# Autodesk Inventor assembly: LifterRight
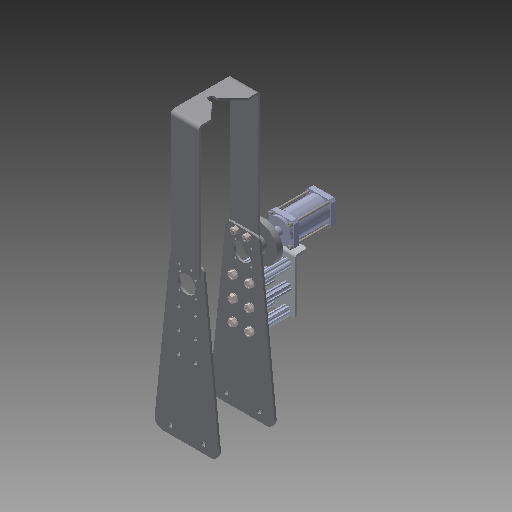
[picture p0: Inventor's stored thumbnail of the model, 512x512]
Saved by Autodesk Inventor 2017 (Build 210142000, 142)
## iProperties
Created: 2017-02-09
Part Number: LifterRight
Document SubType Name: Assembly
Designer: kingb
Author: kingb
## Documents named in this file (10)
- C:\Users\kingb\Desktop\CAD\LifterRight.iam
- C:\Users\kingb\Desktop\CAD\lifterMountMetal.ipt
- C:\Users\kingb\Desktop\CAD\am-2954 AM14U2 2x3 Hole Bracket.ipt
- C:\Users\kingb\Desktop\CAD\am-2878+Banebots+P60+256-11(Fixed).iam
- C:\Users\kingb\Desktop\CAD\newCoupler.ipt
- C:\Users\kingb\Desktop\CAD\Churro 3375.ipt
- C:\Users\kingb\Desktop\CAD\guidebar.ipt
- C:\Users\kingb\Desktop\CAD\10-32x0500_shcs_HX-SHCS 0.19-32x1.375x1-C.ipt
- C:\Users\kingb\Desktop\CAD\FHTS 0.25-20-0.75_FHTS 0.25-20-G-0.75-C.ipt
- C:\Users\kingb\Desktop\CAD\10-32 Nylock Nut.ipt
## Components (30 placed, 9 different names)
1. lifterMountMetal:1 — Mate:5, Mate:6, Insert:12, Insert:14, Insert:15, Insert:16, Insert:17, Insert:26, Insert:27, Mate:11, Mate:12, Mate:13
2. am-2954 AM14U2 2x3 Hole Bracket:1 — Mate:2, Flush:1, Mate:3, Insert:4, Insert:5, Insert:6, Insert:7, Insert:8, Insert:9, Insert:10, Insert:11, Insert:18, Insert:19, Insert:20, Insert:21, Insert:22, Insert:23
3. am-2878+Banebots+P60+256-11(Fixed):1 [sub-assembly] — Mate:2, Flush:1, Mate:3, Angle:2, Mate:13, Mate:14, Mate:15
4. newCoupler:1 — Mate:14, Mate:15
5. Churro 3375:1 — Insert:7
6. Churro 3375:2 — Insert:5
7. Churro 3375:3 — Insert:4, Mate:5
8. Churro 3375:5 — Insert:6
9. guidebar:1 — Mate:6, Angle:2, Insert:24, Insert:25, Insert:28, Insert:29, Mate:11, Mate:12
10. Churro 3375:6 — Insert:9
11. Churro 3375:7 — Insert:8
12. 10-32x0500_shcs_HX-SHCS 0.19-32x1.375x1-C:1 — Insert:10
13. 10-32x0500_shcs_HX-SHCS 0.19-32x1.375x1-C:2 — Insert:11
14. FHTS 0.25-20-0.75_FHTS 0.25-20-G-0.75-C:1 — Insert:20
15. FHTS 0.25-20-0.75_FHTS 0.25-20-G-0.75-C:2 — Insert:21
16. FHTS 0.25-20-0.75_FHTS 0.25-20-G-0.75-C:3 — Insert:23
17. FHTS 0.25-20-0.75_FHTS 0.25-20-G-0.75-C:4 — Insert:22
18. FHTS 0.25-20-0.75_FHTS 0.25-20-G-0.75-C:5 — Insert:18
19. FHTS 0.25-20-0.75_FHTS 0.25-20-G-0.75-C:6 — Insert:19
20. FHTS 0.25-20-0.75_FHTS 0.25-20-G-0.75-C:7 — Insert:16
21. FHTS 0.25-20-0.75_FHTS 0.25-20-G-0.75-C:8 — Insert:17
22. FHTS 0.25-20-0.75_FHTS 0.25-20-G-0.75-C:9 — Insert:14
23. FHTS 0.25-20-0.75_FHTS 0.25-20-G-0.75-C:10 — Insert:15
24. FHTS 0.25-20-0.75_FHTS 0.25-20-G-0.75-C:11
25. FHTS 0.25-20-0.75_FHTS 0.25-20-G-0.75-C:12 — Insert:12
26. 10-32x0500_shcs_HX-SHCS 0.19-32x1.375x1-C:3 — Insert:24
27. 10-32x0500_shcs_HX-SHCS 0.19-32x1.375x1-C:4 — Insert:25
28. 10-32 Nylock Nut:1 — Insert:27
29. 10-32 Nylock Nut:2 — Insert:26
30. lifterMountMetal:2 — Insert:28, Insert:29
## Relationships (36: Insert 25, Mate 9, Flush 1, Angle 1)
- Mate:2: am-2954 AM14U2 2x3 Hole Bracket:1 ↔ am-2878+Banebots+P60+256-11(Fixed):1
- Flush:1 (-6.35 mm): am-2954 AM14U2 2x3 Hole Bracket:1 ↔ am-2878+Banebots+P60+256-11(Fixed):1
- Mate:3: am-2954 AM14U2 2x3 Hole Bracket:1 ↔ am-2878+Banebots+P60+256-11(Fixed):1
- Insert:4: am-2954 AM14U2 2x3 Hole Bracket:1 ↔ Churro 3375:3
- Insert:5: am-2954 AM14U2 2x3 Hole Bracket:1 ↔ Churro 3375:2
- Mate:5: lifterMountMetal:1 ↔ Churro 3375:3
- Insert:6: am-2954 AM14U2 2x3 Hole Bracket:1 ↔ Churro 3375:5
- Insert:7: am-2954 AM14U2 2x3 Hole Bracket:1 ↔ Churro 3375:1
- Mate:6: lifterMountMetal:1 ↔ guidebar:1
- Angle:2 (0 deg): am-2878+Banebots+P60+256-11(Fixed):1 ↔ guidebar:1
- Insert:8: am-2954 AM14U2 2x3 Hole Bracket:1 ↔ Churro 3375:7
- Insert:9: am-2954 AM14U2 2x3 Hole Bracket:1 ↔ Churro 3375:6
- Insert:10: am-2954 AM14U2 2x3 Hole Bracket:1 ↔ 10-32x0500_shcs_HX-SHCS 0.19-32x1.375x1-C:1
- Insert:11: am-2954 AM14U2 2x3 Hole Bracket:1 ↔ 10-32x0500_shcs_HX-SHCS 0.19-32x1.375x1-C:2
- Insert:12: lifterMountMetal:1 ↔ FHTS 0.25-20-0.75_FHTS 0.25-20-G-0.75-C:12
- Insert:14: lifterMountMetal:1 ↔ FHTS 0.25-20-0.75_FHTS 0.25-20-G-0.75-C:9
- Insert:15: lifterMountMetal:1 ↔ FHTS 0.25-20-0.75_FHTS 0.25-20-G-0.75-C:10
- Insert:16: lifterMountMetal:1 ↔ FHTS 0.25-20-0.75_FHTS 0.25-20-G-0.75-C:7
- Insert:17: lifterMountMetal:1 ↔ FHTS 0.25-20-0.75_FHTS 0.25-20-G-0.75-C:8
- Insert:18: am-2954 AM14U2 2x3 Hole Bracket:1 ↔ FHTS 0.25-20-0.75_FHTS 0.25-20-G-0.75-C:5
- Insert:19: am-2954 AM14U2 2x3 Hole Bracket:1 ↔ FHTS 0.25-20-0.75_FHTS 0.25-20-G-0.75-C:6
- Insert:20: am-2954 AM14U2 2x3 Hole Bracket:1 ↔ FHTS 0.25-20-0.75_FHTS 0.25-20-G-0.75-C:1
- Insert:21: am-2954 AM14U2 2x3 Hole Bracket:1 ↔ FHTS 0.25-20-0.75_FHTS 0.25-20-G-0.75-C:2
- Insert:22: am-2954 AM14U2 2x3 Hole Bracket:1 ↔ FHTS 0.25-20-0.75_FHTS 0.25-20-G-0.75-C:4
- Insert:23: am-2954 AM14U2 2x3 Hole Bracket:1 ↔ FHTS 0.25-20-0.75_FHTS 0.25-20-G-0.75-C:3
- Insert:24: guidebar:1 ↔ 10-32x0500_shcs_HX-SHCS 0.19-32x1.375x1-C:3
- Insert:25: guidebar:1 ↔ 10-32x0500_shcs_HX-SHCS 0.19-32x1.375x1-C:4
- Insert:26: lifterMountMetal:1 ↔ 10-32 Nylock Nut:2
- Insert:27: lifterMountMetal:1 ↔ 10-32 Nylock Nut:1
- Insert:28: guidebar:1 ↔ lifterMountMetal:2
- Insert:29: guidebar:1 ↔ lifterMountMetal:2
- Mate:11 (-12.7 mm): lifterMountMetal:1 ↔ guidebar:1
- Mate:12: lifterMountMetal:1 ↔ guidebar:1
- Mate:13: lifterMountMetal:1 ↔ am-2878+Banebots+P60+256-11(Fixed):1
- Mate:14 (12.7 mm): am-2878+Banebots+P60+256-11(Fixed):1 ↔ newCoupler:1
- Mate:15: am-2878+Banebots+P60+256-11(Fixed):1 ↔ newCoupler:1
